# Autodesk Inventor assembly: Ari Tsugi
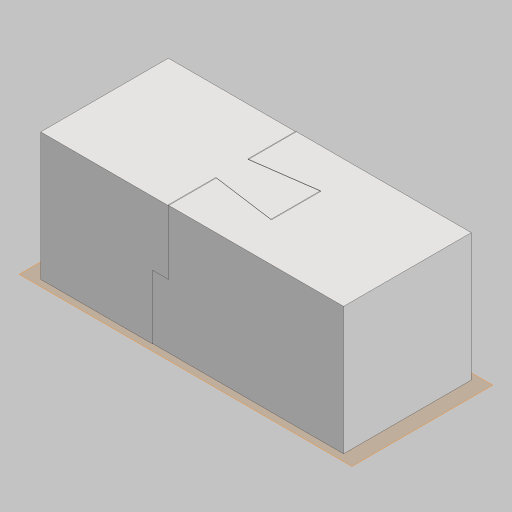
[picture p0: Inventor's stored thumbnail of the model, 512x512]
Saved by Autodesk Inventor 2023 (Build 270158000, 158)
## iProperties
Created: 2026-02-22
Part Number: Ari Tsugi
Document SubType Name: Assembly
Designer: MARTIN MAESTRE
Author: MARTIN MAESTRE
## Documents named in this file (3)
- C:\Users\MARTIN MAESTRE\OneDrive - Universidad de los Andes\POSTGRADO\202610\MAESTRIA\PROBLEMA ESPECIAL\CADS\Fig2\Ari Tsugi.iam
- C:\Users\MARTIN MAESTRE\OneDrive - Universidad de los Andes\POSTGRADO\202610\MAESTRIA\PROBLEMA ESPECIAL\CADS\Fig2\Macho.ipt
- C:\Users\MARTIN MAESTRE\OneDrive - Universidad de los Andes\POSTGRADO\202610\MAESTRIA\PROBLEMA ESPECIAL\CADS\Fig2\Hembra.ipt
## Components (2 placed, 2 different names)
1. Macho:1 — Coincidencia:1, Nivelación:1, Coincidencia:2
2. Hembra:1 — Coincidencia:3
## Relationships (4: Mate 3, Flush 1)
- Coincidencia:1 [Mate]: Macho:1
- Nivelación:1 [Flush]: Macho:1
- Coincidencia:2 [Mate]: Macho:1
- Coincidencia:3 [Mate]: Hembra:1
